# Autodesk Inventor assembly: NewScrewDrive
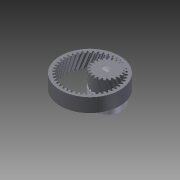
[picture p0: Inventor's stored thumbnail of the model, 180x180]
Saved by Autodesk Inventor 2012 (Build 160160000, 160)
## iProperties
Created: 2011-10-19
Part Number: NewScrewDrive
Document SubType Name: Assembly
Designer: KuttaA
Author: KuttaA
## Documents named in this file (4)
- C:\Users\KuttaA\Dropbox\Hexapod Research\Leg Design\Other Parts\inter\NewScrewDrive.iam
- C:\Users\KuttaA\Dropbox\Hexapod Research\Leg Design\Other Parts\inter\MotorToGear.ipt
- C:\Users\KuttaA\Dropbox\Hexapod Research\Leg Design\Other Parts\inter\GearToScrew.ipt
- C:\Users\KuttaA\Dropbox\Hexapod Research\Leg Design\Other Parts\inter\NewScrewDrive\Design Accelerator\Spur Gears2.iam
## Components (3 placed, 3 different names)
1. MotorToGear:1 — Mate:3, Rotation:1, Angle:2, Mate:4, Mate:1, Mate:7, Tangent:1
2. GearToScrew:1 — Rotation:1, Angle:2, Mate:1, Mate:5, Mate:8, Mate:9
3. Spur Gears:1 [sub-assembly] — Mate:5, Mate:7, Mate:8, Tangent:1, Mate:9
## Relationships (10: Mate 7, RelateRotation 1, Angle 1, Tangent 1)
- Mate:3: MotorToGear:1
- Rotation:1 [RelateRotation] (0.5 ul): MotorToGear:1 ↔ GearToScrew:1
- Angle:2 (180 deg): MotorToGear:1 ↔ GearToScrew:1
- Mate:4: MotorToGear:1
- Mate:1: MotorToGear:1 ↔ GearToScrew:1
- Mate:5: GearToScrew:1 ↔ Spur Gears:1
- Mate:7: MotorToGear:1 ↔ Spur Gears:1
- Mate:8: GearToScrew:1 ↔ Spur Gears:1
- Tangent:1: MotorToGear:1 ↔ Spur Gears:1
- Mate:9: GearToScrew:1 ↔ Spur Gears:1
